# Autodesk Inventor assembly: Marco_apm_003-2
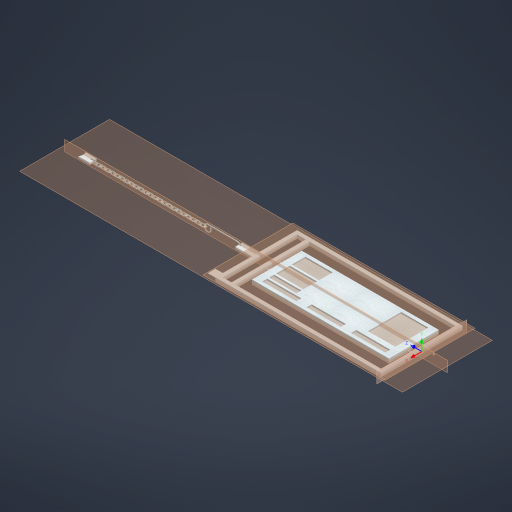
[picture p0: Inventor's stored thumbnail of the model, 512x512]
Saved by Autodesk Inventor 2024 (Build 280153000, 153)
## iProperties
Created: 2023-05-17
Part Number: Marco_apm_003-2
Document SubType Name: Assembly
Designer: javie
Author: javie
## Documents named in this file (6)
- C:\Users\javie\Downloads\Piezas CMR\Marco_APM_003\Marco_apm_003-2.iam
- C:\Users\javie\Downloads\Piezas CMR\Marco_Conveyor_Aereo.iam
- C:\Users\javie\Downloads\Piezas CMR\Marcos_solids\S_horizontal.ipt
- C:\Users\javie\Downloads\Piezas CMR\Marco_APM_003\Piezas\APM_003-2.ipt
- C:\Users\javie\Downloads\Piezas CMR\Marcos_solids\Topes_apm_002-2.ipt
- C:\Users\javie\Downloads\Piezas CMR\Marcos_solids\1000.ipt
## Components (6 placed, 5 different names)
1. Marco_Conveyor_Aereo:1 [sub-assembly] — Insertar:7, Insertar:8, Nivelación:1, Nivelación:2
2. APM_003-2:2 — Insertar:9, Insertar:10, Insertar:13, Insertar:14
3. Topes_apm_002-2:2 — Insertar:7, Insertar:8, Insertar:13, Insertar:14
4. S_horizontal:1 — Insertar:11, Insertar:12
5. Topes_apm_002-2:3 — Insertar:9, Insertar:10, Insertar:11, Insertar:12
6. 1000:1 — Nivelación:1, Nivelación:2
## Relationships (10: Insert 8, Flush 2)
- Insertar:7: Marco_Conveyor_Aereo:1 ↔ Topes_apm_002-2:2
- Insertar:8: Marco_Conveyor_Aereo:1 ↔ Topes_apm_002-2:2
- Insertar:9: APM_003-2:2 ↔ Topes_apm_002-2:3
- Insertar:10: APM_003-2:2 ↔ Topes_apm_002-2:3
- Insertar:11: S_horizontal:1 ↔ Topes_apm_002-2:3
- Insertar:12: S_horizontal:1 ↔ Topes_apm_002-2:3
- Insertar:13: APM_003-2:2 ↔ Topes_apm_002-2:2
- Insertar:14: APM_003-2:2 ↔ Topes_apm_002-2:2
- Nivelación:1 [Flush]: Marco_Conveyor_Aereo:1 ↔ 1000:1
- Nivelación:2 [Flush]: Marco_Conveyor_Aereo:1 ↔ 1000:1
